# Autodesk Inventor assembly: UpperArmActuatorShaft
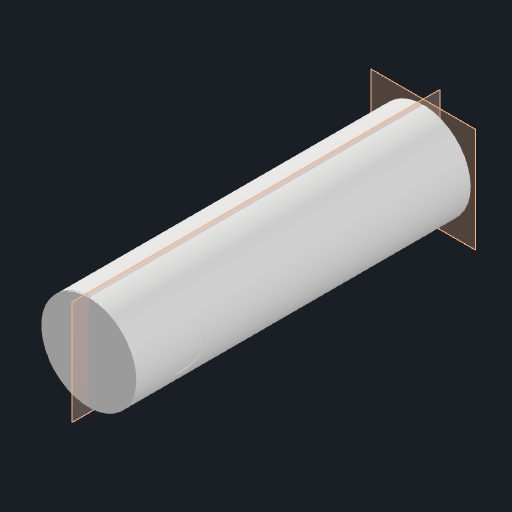
[picture p0: Inventor's stored thumbnail of the model, 512x512]
Saved by Autodesk Inventor 2023 (Build 270158000, 158)
## iProperties
Created: 2023-03-23
Part Number: UpperArmActuatorShaft
Document SubType Name: Assembly
Designer: Val
Author: Val
## Documents named in this file (3)
- C:\Users\valer\Desktop\str1ker\cad\external\UpperArmActuator\UpperArmActuatorShaft.iam
- C:\Users\valer\Desktop\str1ker\cad\external\UpperArmActuator\UpperArmActuatorShaft.ipt
- C:\Users\valer\Desktop\str1ker\cad\external\UpperArmActuator\UpperArmActuatorShaftBoundingBox.ipt
## Components (2 placed, 2 different names)
1. UpperArmActuatorShaft:1 — Mate:1, Mate:2, Flush:1, Mate:3
2. UpperArmActuatorShaftBoundingBox:1 — Flush:2, Flush:3, Flush:4
## Relationships (7: Flush 4, Mate 3)
- Mate:1: UpperArmActuatorShaft:1
- Mate:2: UpperArmActuatorShaft:1
- Flush:1: UpperArmActuatorShaft:1
- Flush:2: UpperArmActuatorShaftBoundingBox:1
- Flush:3: UpperArmActuatorShaftBoundingBox:1
- Flush:4: UpperArmActuatorShaftBoundingBox:1
- Mate:3: UpperArmActuatorShaft:1
